# Autodesk Inventor assembly: Assembly1
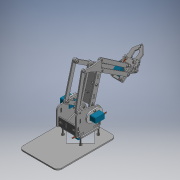
[picture p0: Inventor's stored thumbnail of the model, 180x180]
Saved by Autodesk Inventor 2019.2 (Build 232265000, 265)
## iProperties
Part Number: Assembly1
Document SubType Name: Assembly
Designer: richard.girt
Mass: 166.526 g
Surface Area: 1092.64 cm^2
Volume: 130.588 cm^3
Density: 1.2752 g/cm^3
Author: richard.girt
## Documents named in this file (18)
- C:\Users\richard.girt\Desktop\2 Axis robotic arm\Assembly1.iam
- C:\Users\richard.girt\Desktop\2 Axis robotic arm\Part1.ipt
- C:\Users\richard.girt\Desktop\2 Axis robotic arm\Part3.ipt
- C:\Users\richard.girt\Desktop\2 Axis robotic arm\Part4.ipt
- C:\Users\richard.girt\Desktop\2 Axis robotic arm\Part7.ipt
- C:\Users\richard.girt\Desktop\2 Axis robotic arm\Part8.ipt
- C:\Users\richard.girt\Desktop\2 Axis robotic arm\SG90.ipt
- C:\Users\richard.girt\Desktop\2 Axis robotic arm\Assembly2.iam
- C:\Users\richard.girt\Desktop\2 Axis robotic arm\Assembly3.iam
- C:\Users\richard.girt\Desktop\2 Axis robotic arm\Part16.ipt
- C:\Users\richard.girt\Desktop\2 Axis robotic arm\Assembly4.iam
- C:\Users\richard.girt\Desktop\2 Axis robotic arm\Part26.ipt
- C:\Users\richard.girt\Desktop\2 Axis robotic arm\ANSI B 18.2.4.1 M - M3 x 0.5Style 1.ipt
- C:\Users\richard.girt\Desktop\2 Axis robotic arm\ANSI B18.3.4M - M3 x 0.5 x 8(1).ipt
- C:\Users\richard.girt\Documents\Inventor\Content Center Files\R2019\en-US\ANSI B18.3.4M(2)\ANSI B18.3.4M - M3 x 0.5 x 20(1).ipt
- C:\Users\richard.girt\Desktop\2 Axis robotic arm\Assembly5.iam
- C:\Users\richard.girt\Desktop\2 Axis robotic arm\Part24.ipt
- C:\_Vault\Content Center\en-US\ANSI B18.3.4M(2)\ANSI B18.3.4M - M3 x 0.5 x 6(1).ipt
## Components (37 placed, 17 different names)
1. Part7:1 — Flush:2, Mate:8, Rigid:11, Rigid:16, Rigid:17, Rigid:18
2. Part1:2 — Mate:2, Mate:3, Mate:4, Rigid:9, Rigid:10
3. Part3:1 — Mate:15, Mate:18, Mate:19
4. Part4:2 — Mate:12, Mate:13, Mate:27, Rotational:14, Rigid:21
5. Part4:3 — Cylindrical:4, Mate:25, Flush:3, Mate:26, Rigid:20, Rigid:27
6. Part8:1 — Mate:5, Mate:6, Flush:1, Mate:8
7. SG90:1 — Mate:2, Mate:3, Mate:4, Mate:5, Mate:6, Flush:1, Flush:2, Mate:7, Rigid:7
8. Assembly2:1 [sub-assembly] — Mate:11, Mate:14, Rotational:11, Mate:20, Rotational:15, Rigid:23
9. Assembly3:1 [sub-assembly] — Rigid:7, Mate:12, Rotational:10, Rotational:11, Rotational:12, Rigid:24
10. Part16:1 — Cylindrical:4, Mate:10, Mate:13, Mate:26, Mate:27
11. Part26:1 — Mate:14, Mate:15, Mate:21, Mate:22, Mate:23, Rotational:13, Rigid:22, Rigid:25
12. Part4:4 — Mate:10, Mate:11, Mate:20, Mate:21, Mate:24, Flush:3, Rigid:26
13. ANSI B18.3.4M - M3 x 0.5 x 8(1):1 — Rigid:9
14. ANSI B18.3.4M - M3 x 0.5 x 8(1):2 — Rigid:10
15. ANSI B 18.2.4.1 M - M3 x 0.5Style 1:1 — Rigid:12
16. ANSI B 18.2.4.1 M - M3 x 0.5Style 1:2
17. ANSI B 18.2.4.1 M - M3 x 0.5Style 1:3
18. ANSI B 18.2.4.1 M - M3 x 0.5Style 1:4
19. Assembly5:1 [sub-assembly] — Rotational:10, Mate:18, Mate:19, Rigid:19
20. Assembly4:1 [sub-assembly] — Mate:22, Mate:23, Mate:24, Mate:25
21. Part24:1 — Rotational:12
22. Part24:2 — Rotational:13
23. ANSI B18.3.4M - M3 x 0.5 x 8(1):3 — Rotational:14
24. ANSI B18.3.4M - M3 x 0.5 x 8(1):4 — Rotational:15
25. ANSI B18.3.4M - M3 x 0.5 x 8(1):5 — Rigid:22
26. ANSI B18.3.4M - M3 x 0.5 x 8(1):6 — Rigid:25
27. ANSI B18.3.4M - M3 x 0.5 x 8(1):7 — Rigid:26
28. ANSI B18.3.4M - M3 x 0.5 x 8(1):8 — Rigid:27
29. Forged Hexagon Socket Button Head Cap Screw - Metric M3 x 0.5 x 6:1 — Rigid:19
30. Forged Hexagon Socket Button Head Cap Screw - Metric M3 x 0.5 x 6:2 — Rigid:21
31. Forged Hexagon Socket Button Head Cap Screw - Metric M3 x 0.5 x 6:3 — Rigid:20
32. Forged Hexagon Socket Button Head Cap Screw - Metric M3 x 0.5 x 6:4 — Rigid:23
33. Forged Hexagon Socket Button Head Cap Screw - Metric M3 x 0.5 x 6:5 — Rigid:24
34. Forged Hexagon Socket Button Head Cap Screw - Metric M3 x 0.5 x 20:3 — Rigid:17
35. Forged Hexagon Socket Button Head Cap Screw - Metric M3 x 0.5 x 20:2 — Rigid:18
36. Forged Hexagon Socket Button Head Cap Screw - Metric M3 x 0.5 x 20:1 — Rigid:11, Rigid:12
37. Forged Hexagon Socket Button Head Cap Screw - Metric M3 x 0.5 x 20:4 — Rigid:16
## Relationships (53: Mate 23, WeldJoint 20, RevoluteJoint 6, Flush 3, CylindricalJoint 1)
- Mate:2: Part1:2 ↔ SG90:1
- Mate:3: Part1:2 ↔ SG90:1
- Mate:4: Part1:2 ↔ SG90:1
- Mate:5: Part8:1 ↔ SG90:1
- Mate:6: Part8:1 ↔ SG90:1
- Flush:1: Part8:1 ↔ SG90:1
- Flush:2: Part7:1 ↔ SG90:1
- Mate:7: SG90:1
- Mate:8: Part7:1 ↔ Part8:1
- Rigid:7 [WeldJoint]: SG90:1 ↔ Assembly3:1
- Cylindrical:4: Part4:3 ↔ Part16:1
- Mate:10: Part16:1 ↔ Part4:4
- Mate:11: Assembly2:1 ↔ Part4:4
- Mate:12: Part4:2 ↔ Assembly3:1
- Mate:13: Part4:2 ↔ Part16:1
- Mate:14: Assembly2:1 ↔ Part26:1
- Mate:15: Part3:1 ↔ Part26:1
- Rigid:9 [WeldJoint]: Part1:2 ↔ ANSI B18.3.4M - M3 x 0.5 x 8(1):1
- Rigid:10 [WeldJoint]: Part1:2 ↔ ANSI B18.3.4M - M3 x 0.5 x 8(1):2
- Rigid:11 [WeldJoint]: Part7:1 ↔ Forged Hexagon Socket Button Head Cap Screw - Metric M3 x 0.5 x 20:1
- Rigid:12 [WeldJoint] (2.8 mm): ANSI B 18.2.4.1 M - M3 x 0.5Style 1:1 ↔ Forged Hexagon Socket Button Head Cap Screw - Metric M3 x 0.5 x 20:1
- [WeldJoint] (2.8 mm): ANSI B 18.2.4.1 M - M3 x 0.5Style 1:2 ↔ Forged Hexagon Socket Button Head Cap Screw - Metric M3 x 0.5 x 20:2
- [WeldJoint] (2.8 mm): ANSI B 18.2.4.1 M - M3 x 0.5Style 1:3 ↔ Forged Hexagon Socket Button Head Cap Screw - Metric M3 x 0.5 x 20:3
- [WeldJoint] (2.8 mm): ANSI B 18.2.4.1 M - M3 x 0.5Style 1:4 ↔ Forged Hexagon Socket Button Head Cap Screw - Metric M3 x 0.5 x 20:4
- Rigid:16 [WeldJoint]: Part7:1 ↔ Forged Hexagon Socket Button Head Cap Screw - Metric M3 x 0.5 x 20:4
- Rigid:17 [WeldJoint]: Part7:1 ↔ Forged Hexagon Socket Button Head Cap Screw - Metric M3 x 0.5 x 20:3
- Rigid:18 [WeldJoint]: Part7:1 ↔ Forged Hexagon Socket Button Head Cap Screw - Metric M3 x 0.5 x 20:2
- Rotational:10 [RevoluteJoint]: Assembly3:1 ↔ Assembly5:1
- Mate:18: Part3:1 ↔ Assembly5:1
- Mate:19 (0.1 mm): Part3:1 ↔ Assembly5:1
- Rotational:11 [RevoluteJoint]: Assembly2:1 ↔ Assembly3:1
- Mate:20 (0.1 mm): Assembly2:1 ↔ Part4:4
- Mate:21: Part26:1 ↔ Part4:4
- Mate:22: Part26:1 ↔ Assembly4:1
- Mate:23 (0.1 mm): Part26:1 ↔ Assembly4:1
- Mate:24 (0.1 mm): Part4:4 ↔ Assembly4:1
- Mate:25: Part4:3 ↔ Assembly4:1
- Flush:3: Part4:3 ↔ Part4:4
- Mate:26 (0.1 mm): Part4:3 ↔ Part16:1
- Mate:27 (0.1 mm): Part4:2 ↔ Part16:1
- Rotational:12 [RevoluteJoint] (-0.1 mm): Assembly3:1 ↔ Part24:1
- Rotational:13 [RevoluteJoint] (-0.1 mm): Part26:1 ↔ Part24:2
- Rigid:19 [WeldJoint]: Assembly5:1 ↔ Forged Hexagon Socket Button Head Cap Screw - Metric M3 x 0.5 x 6:1
- Rotational:14 [RevoluteJoint]: Part4:2 ↔ ANSI B18.3.4M - M3 x 0.5 x 8(1):3
- Rigid:20 [WeldJoint]: Part4:3 ↔ Forged Hexagon Socket Button Head Cap Screw - Metric M3 x 0.5 x 6:3
- Rigid:21 [WeldJoint]: Part4:2 ↔ Forged Hexagon Socket Button Head Cap Screw - Metric M3 x 0.5 x 6:2
- Rotational:15 [RevoluteJoint]: Assembly2:1 ↔ ANSI B18.3.4M - M3 x 0.5 x 8(1):4
- Rigid:22 [WeldJoint]: Part26:1 ↔ ANSI B18.3.4M - M3 x 0.5 x 8(1):5
- Rigid:23 [WeldJoint]: Assembly2:1 ↔ Forged Hexagon Socket Button Head Cap Screw - Metric M3 x 0.5 x 6:4
- Rigid:24 [WeldJoint]: Assembly3:1 ↔ Forged Hexagon Socket Button Head Cap Screw - Metric M3 x 0.5 x 6:5
- Rigid:25 [WeldJoint]: Part26:1 ↔ ANSI B18.3.4M - M3 x 0.5 x 8(1):6
- Rigid:26 [WeldJoint]: Part4:4 ↔ ANSI B18.3.4M - M3 x 0.5 x 8(1):7
- Rigid:27 [WeldJoint] (-1.1 mm): Part4:3 ↔ ANSI B18.3.4M - M3 x 0.5 x 8(1):8
## Named parameters: d100_d99 = 2.8 mm, d101_d99 = 2.8 mm, d102_d99 = 2.8 mm
